# Autodesk Inventor assembly: Segment_Small_Ass
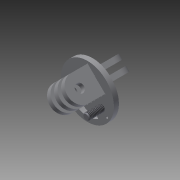
[picture p0: Inventor's stored thumbnail of the model, 180x180]
Saved by Autodesk Inventor 2014 SP1 (Build 180222100, 222)
## iProperties
Created: 2014-03-20
Part Number: Segment_Small_Ass
Document SubType Name: Assembly
Designer: ehagerup
Author: ehagerup
## Documents named in this file (5)
- C:\Users\ehagerup\SkyDrive\Documents\Mechanical Sketches\Animatronic Tail V4\Segment_Small_Ass.iam
- C:\Users\ehagerup\SkyDrive\Documents\Mechanical Sketches\Animatronic Tail V4\Segment_Small.ipt
- C:\Users\ehagerup\SkyDrive\Documents\Mechanical Sketches\Animatronic Tail V4\Connector_3.ipt
- C:\Users\ehagerup\SkyDrive\Documents\Mechanical Sketches\Animatronic Tail V4\Connector_2.ipt
- C:\Users\ehagerup\Documents\Inventor\Content Center Files\R2014\en-US\JIS B 1180  A+B\JIS B 1180 - A + B M4x12x5.88 - 10.ipt
## Components (8 placed, 4 different names)
1. Segment_Small:1 — Flush:7, Mate:1, Mate:2, Mate:3, Flush:8, Mate:4, Mate:5, Mate:6, Mate:7, Mate:8, Mate:9, Mate:10, Mate:11
2. Connector_3:1 — Flush:1, Flush:6, Flush:7, Mate:1, Mate:2
3. Connector_3:2 — Flush:1, Flush:6, Mate:3
4. Connector_2:1 — Flush:3, Flush:4, Mate:7
5. Connector_2:2 — Flush:2, Flush:3, Flush:4, Flush:5, Mate:6
6. Connector_2:3 — Flush:2, Flush:5, Flush:8, Mate:4, Mate:5
7. JIS B 1180 A+B - Metric A + B M4x12:1 — Mate:8, Mate:9
8. JIS B 1180 A+B - Metric A + B M4x12:2 — Mate:10, Mate:11
## Relationships (19: Mate 11, Flush 8)
- Flush:1: Connector_3:1 ↔ Connector_3:2
- Flush:2: Connector_2:2 ↔ Connector_2:3
- Flush:3: Connector_2:1 ↔ Connector_2:2
- Flush:4: Connector_2:1 ↔ Connector_2:2
- Flush:5: Connector_2:2 ↔ Connector_2:3
- Flush:6: Connector_3:1 ↔ Connector_3:2
- Flush:7: Segment_Small:1 ↔ Connector_3:1
- Mate:1: Segment_Small:1 ↔ Connector_3:1
- Mate:2: Segment_Small:1 ↔ Connector_3:1
- Mate:3: Segment_Small:1 ↔ Connector_3:2
- Flush:8: Segment_Small:1 ↔ Connector_2:3
- Mate:4: Segment_Small:1 ↔ Connector_2:3
- Mate:5: Segment_Small:1 ↔ Connector_2:3
- Mate:6: Segment_Small:1 ↔ Connector_2:2
- Mate:7: Segment_Small:1 ↔ Connector_2:1
- Mate:8: Segment_Small:1 ↔ JIS B 1180 A+B - Metric A + B M4x12:1
- Mate:9: Segment_Small:1 ↔ JIS B 1180 A+B - Metric A + B M4x12:1
- Mate:10: Segment_Small:1 ↔ JIS B 1180 A+B - Metric A + B M4x12:2
- Mate:11: Segment_Small:1 ↔ JIS B 1180 A+B - Metric A + B M4x12:2
